# Autodesk Inventor assembly: Output Link
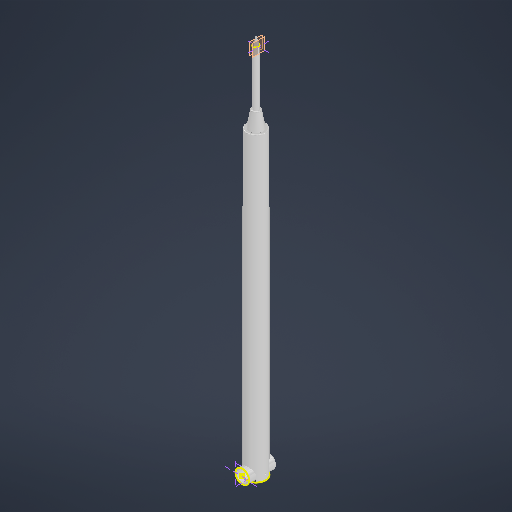
[picture p0: Inventor's stored thumbnail of the model, 512x512]
Saved by Autodesk Inventor 2026.3 (Build 303398000, 398)
## iProperties
Created: 2026-07-24
Part Number: Output Link
Document SubType Name: Assembly
Designer: matot
Author: matot
## Documents named in this file (5)
- C:\Users\matot\OneDrive - Stellenbosch University\2026\MechatronicsProject478\Building the joint\Joint Assembly\Output Link.iam
- C:\Users\matot\OneDrive - Stellenbosch University\2026\MechatronicsProject478\Building the joint\Joint Assembly\Output lint interface cuff.ipt
- C:\Users\matot\OneDrive - Stellenbosch University\2026\MechatronicsProject478\Building the joint\Joint Assembly\Output link body.ipt
- C:\Users\matot\OneDrive - Stellenbosch University\2026\MechatronicsProject478\Building the joint\Joint Assembly\Output link probe hub.ipt
- C:\Users\matot\OneDrive - Stellenbosch University\2026\MechatronicsProject478\Building the joint\Joint Assembly\Output link probe.ipt
## Components (4 placed, 4 different names)
1. Output lint interface cuff:1 — Mate:1, Mate:2
2. Output link body:1 — Mate:1, Mate:2, Insert:1
3. Output link probe hub:1 — Insert:1, Insert:2
4. Output link probe:1 — Insert:2
## Relationships (4: Mate 2, Insert 2)
- Mate:1: Output lint interface cuff:1 ↔ Output link body:1
- Mate:2: Output lint interface cuff:1 ↔ Output link body:1
- Insert:1: Output link body:1 ↔ Output link probe hub:1
- Insert:2 (-100 mm): Output link probe hub:1 ↔ Output link probe:1
